# Autodesk Inventor assembly: Microswitch - Omron SS-01GL2-E
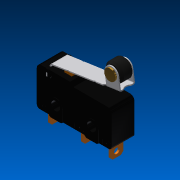
[picture p0: Inventor's stored thumbnail of the model, 180x180]
Saved by Autodesk Inventor 2013 (Build 170138000, 138)
## iProperties
Created: 2012-05-23
Document SubType Name: Assembly
Designer: sdarley
Project: Microswitch - Omron SS-01GL2-E
Catalog Web Link: http://australia.rs-online.com/web/p/microswitches/6822629/
Description: Microswitch - Omron SS-01GL2-E
Vendor: Omron
Stock Number: SS-01GL2-E
Author: sdarley
Title: Microswitch - Omron SS-01GL2-E
Revision Number: 1
## Documents named in this file (7)
- C:\Users\sdarley\Documents\Inventor\General Design Work\Microswitch - Omron SS-01GL2-E\Microswitch - Omron SS-01GL2-E.iam
- C:\Users\sdarley\Documents\Inventor\General Design Work\Microswitch - Omron SS-01GL2-E\Components\Omron SS-01GL2-E Microswitch Housing.ipt
- C:\Users\sdarley\Documents\Inventor\General Design Work\Microswitch - Omron SS-01GL2-E\Components\Omron SS-01GL2-E Microswitch Contact.ipt
- C:\Users\sdarley\Documents\Inventor\General Design Work\Microswitch - Omron SS-01GL2-E\Components\Omron SS-01GL2-E Microswitch Button.ipt
- C:\Users\sdarley\Documents\Inventor\General Design Work\Microswitch - Omron SS-01GL2-E\Components\Omron SS-01GL2-E Microswitch Spring Lever.ipt
- C:\Users\sdarley\Documents\Inventor\General Design Work\Microswitch - Omron SS-01GL2-E\Components\Omron SS-01GL2-E Microswitch Roller Pin.ipt
- C:\Users\sdarley\Documents\Inventor\General Design Work\Microswitch - Omron SS-01GL2-E\Components\Omron SS-01GL2-E Microswitch Roller.ipt
## Components (8 placed, 6 different names)
1. Omron SS-01GL2-E Microswitch Housing:1 — Flush:1, Flush:2, Flush:3, Flush:4, Mate:1, Flush:5, Mate:2, Mate:3, Mate:4, Mate:5, Flush:8, Mate:6, Mate:7, Flush:9, Mate:8, Flush:10, Mate:11
2. Omron SS-01GL2-E Microswitch Button:1 — Flush:8, Mate:6, Mate:7
3. Omron SS-01GL2-E Microswitch Spring Lever:1 — Flush:9, Mate:8, Flush:10, Flush:11, Mate:9
4. Omron SS-01GL2-E Microswitch Roller Pin:1 — Flush:11, Mate:9, Mate:10
5. Omron SS-01GL2-E Microswitch Roller:1 — Mate:10, Mate:11
6. Omron SS-01GL2-E Microswitch Contact:1 — Flush:4, Mate:1, Flush:5, Flush:6
7. Omron SS-01GL2-E Microswitch Contact:2 — Mate:3, Mate:4, Flush:6, Flush:7
8. Omron SS-01GL2-E Microswitch Contact:3 — Mate:2, Mate:5, Flush:7
## Relationships (22: Flush 11, Mate 11)
- Flush:1: Omron SS-01GL2-E Microswitch Housing:1
- Flush:2: Omron SS-01GL2-E Microswitch Housing:1
- Flush:3: Omron SS-01GL2-E Microswitch Housing:1
- Flush:4: Omron SS-01GL2-E Microswitch Housing:1 ↔ Omron SS-01GL2-E Microswitch Contact:1
- Mate:1: Omron SS-01GL2-E Microswitch Housing:1 ↔ Omron SS-01GL2-E Microswitch Contact:1
- Flush:5 (-1.6 mm): Omron SS-01GL2-E Microswitch Housing:1 ↔ Omron SS-01GL2-E Microswitch Contact:1
- Mate:2: Omron SS-01GL2-E Microswitch Housing:1 ↔ Omron SS-01GL2-E Microswitch Contact:3
- Mate:3: Omron SS-01GL2-E Microswitch Housing:1 ↔ Omron SS-01GL2-E Microswitch Contact:2
- Mate:4: Omron SS-01GL2-E Microswitch Housing:1 ↔ Omron SS-01GL2-E Microswitch Contact:2
- Mate:5: Omron SS-01GL2-E Microswitch Housing:1 ↔ Omron SS-01GL2-E Microswitch Contact:3
- Flush:6 (8.8 mm): Omron SS-01GL2-E Microswitch Contact:1 ↔ Omron SS-01GL2-E Microswitch Contact:2
- Flush:7 (7.3 mm): Omron SS-01GL2-E Microswitch Contact:2 ↔ Omron SS-01GL2-E Microswitch Contact:3
- Flush:8: Omron SS-01GL2-E Microswitch Housing:1 ↔ Omron SS-01GL2-E Microswitch Button:1
- Mate:6: Omron SS-01GL2-E Microswitch Housing:1 ↔ Omron SS-01GL2-E Microswitch Button:1
- Mate:7: Omron SS-01GL2-E Microswitch Housing:1 ↔ Omron SS-01GL2-E Microswitch Button:1
- Flush:9: Omron SS-01GL2-E Microswitch Housing:1 ↔ Omron SS-01GL2-E Microswitch Spring Lever:1
- Mate:8: Omron SS-01GL2-E Microswitch Housing:1 ↔ Omron SS-01GL2-E Microswitch Spring Lever:1
- Flush:10: Omron SS-01GL2-E Microswitch Housing:1 ↔ Omron SS-01GL2-E Microswitch Spring Lever:1
- Flush:11: Omron SS-01GL2-E Microswitch Spring Lever:1 ↔ Omron SS-01GL2-E Microswitch Roller Pin:1
- Mate:9: Omron SS-01GL2-E Microswitch Spring Lever:1 ↔ Omron SS-01GL2-E Microswitch Roller Pin:1
- Mate:10: Omron SS-01GL2-E Microswitch Roller Pin:1 ↔ Omron SS-01GL2-E Microswitch Roller:1
- Mate:11: Omron SS-01GL2-E Microswitch Housing:1 ↔ Omron SS-01GL2-E Microswitch Roller:1
